# Autodesk Inventor assembly: halfdrawerassem
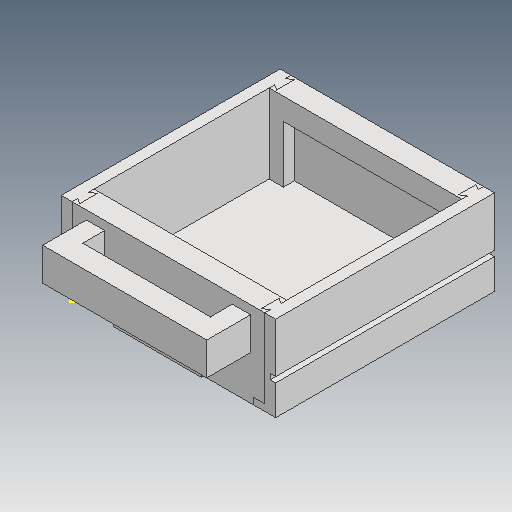
[picture p0: Inventor's stored thumbnail of the model, 512x512]
Saved by Autodesk Inventor 2025.2 (Build 292293000, 293)
## iProperties
Created: 2025-02-25
Part Number: halfdrawerassem
Document SubType Name: Assembly
Designer: email
Author: email
## Documents named in this file (3)
- C:\Users\email\Desktop\Projects\modularboxes\V1\halfdrawerassem.iam
- C:\Users\email\Desktop\Projects\modularboxes\V1\drawersidehalf.ipt
- C:\Users\email\Desktop\Projects\modularboxes\V1\maindrawerhalf.ipt
## Components (3 placed, 2 different names)
1. drawersidehalf:1
2. maindrawerhalf:1
3. drawersidehalf:2
## Relationships (6: Mate 6)
- [Mate]: drawersidehalf:1 ↔ maindrawerhalf:1
- [Mate]: drawersidehalf:1 ↔ maindrawerhalf:1
- [Mate]: drawersidehalf:1 ↔ maindrawerhalf:1
- [Mate]: maindrawerhalf:1 ↔ drawersidehalf:2
- [Mate]: maindrawerhalf:1 ↔ drawersidehalf:2
- [Mate]: maindrawerhalf:1 ↔ drawersidehalf:2
